# Autodesk Inventor assembly: bottom_cover
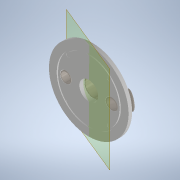
[picture p0: Inventor's stored thumbnail of the model, 180x180]
Saved by Autodesk Inventor 2021 (Build 250183000, 183)
## iProperties
Created: 2024-02-20
Part Number: bottom_cover
Document SubType Name: Assembly
Designer: Sebastián
Author: Sebastián
## Documents named in this file (5)
- C:\Users\Sebastián\Documents\Inventor\PLD SAP\bottom_cover.iam
- C:\Users\Sebastián\Documents\Inventor\PLD SAP\KF160.ipt
- C:\Users\Sebastián\Documents\Inventor\PLD_Chamber\Hositrad_KF40-44.5-30.ipt
- C:\Users\Sebastián\Documents\Inventor\PLD_Chamber\Hositrad_KF25-25-40.ipt
- C:\Users\Sebastián\Documents\Inventor\PLD SAP\KF25-40_angled.ipt
## Components (4 placed, 4 different names)
1. KF160:1 — Rotational:1, Rotational:2, Rigid:1
2. Hositrad_KF40-44.5-30:1 — Rotational:1
3. Hositrad_KF25-25-40:1 — Rotational:2
4. KF25-40_angled:1 — Rigid:1
## Relationships (3: RevoluteJoint 2, WeldJoint 1)
- Rotational:1 [RevoluteJoint]: KF160:1 ↔ Hositrad_KF40-44.5-30:1
- Rotational:2 [RevoluteJoint]: KF160:1 ↔ Hositrad_KF25-25-40:1
- Rigid:1 [WeldJoint]: KF160:1 ↔ KF25-40_angled:1
